# Autodesk Inventor assembly: M12CamMirror
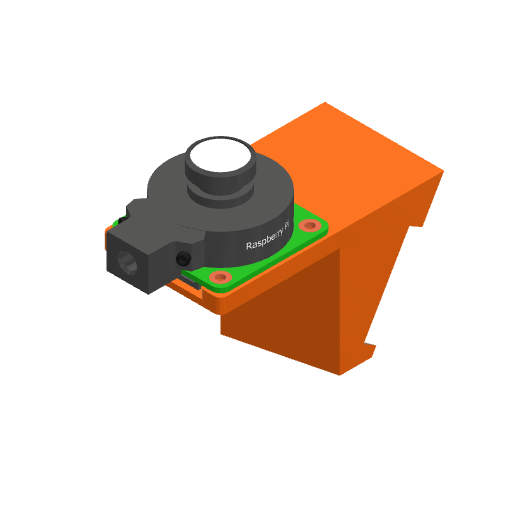
[picture p0: Inventor's stored thumbnail of the model, 512x512]
Saved by Autodesk Inventor 2025.2 (Build 292293000, 293)
## iProperties
Created: 2026-05-15
Part Number: M12CamMirror
Document SubType Name: Assembly
Designer: rolan
Author: rolan
## Documents named in this file (3)
- C:\Users\rolan\Documents\PhD\Inventor\Assembly\M12CamMirror.iam
- C:\Users\rolan\Documents\PhD\Inventor\3D Files\raspberry-pi-hq-camera-m12-fisheye-lens-1.snapshot.1\RPiHQCameraM12\RPiHQCameraM12\RPiHQCameraM12.ipt
- C:\Users\rolan\Documents\PhD\Inventor\Parts\CameraMountM12Mirror.ipt
## Components (2 placed, 2 different names)
1. RPiHQCameraM12:1 — Mate:1, Mate:2, Mate:3
2. CameraMountM12Mirror:1 — Mate:1, Mate:2, Mate:3
## Relationships (3: Mate 3)
- Mate:1: RPiHQCameraM12:1 ↔ CameraMountM12Mirror:1
- Mate:2: RPiHQCameraM12:1 ↔ CameraMountM12Mirror:1
- Mate:3: RPiHQCameraM12:1 ↔ CameraMountM12Mirror:1
